# Autodesk Inventor assembly: WA673SA
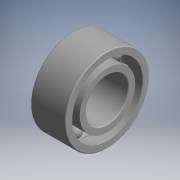
[picture p0: Inventor's stored thumbnail of the model, 180x180]
Saved by Autodesk Inventor 2017.3 (Build 213256000, 256)
## iProperties
Category: PARTsolutions
Company: NTN
Part Number: WA673SA
Catalog Web Link: www.cadenas.de
Description: With single shield Z-
Vendor: NTN
Document SubType Name: Assembly
Designer: partserver
Manufacturer: NTN
Mass: 0.0350333 g
Surface Area: 2.11591 cm^2
Volume: 0.0350333 cm^3
Density: 1 g/cm^3
Title: WA673SA
Author: Cadenas PARTsolutions
PSOL_IDENT_0: {$CADENAS_DATA\23d-libs\ntn\ball_roller_bearings\miniature_extra_small_bb\metric_system_sizes\mss_z_
PSOL_IDENT_1: asmtab.prj},185 {VTYP=3D},{STYP=ASSTAB},{NB=WA673SA},{LINA=WA673SA},{NN=With single shield Z},{DATE=
PSOL_IDENT_2: 21.12.2021 04:23:05},{GEOMDATE=10.03.2020 01:12:32},{VERSION=},{LINEID=11430},{WBVAR=},{WBNUMERIC=}
PSOL_IDENT_3: {NB=WA673SA},{LINA=WA673SA},{KT=DUMMY},{IDNR=},{SD=3.0},{D=6},{B=2.0},{B1=2.5},{D1=7.2},{D2=7.2},{C
PSOL_IDENT_4: 1=0.6},{C2=0.6},{R=0.08},{ORDER=WA673SA},{CR=268},{COR=94},{CU=2.47},{CRF=25},{CORF=9,5},{LSG=60 000
PSOL_IDENT_5: },{LSO=71 000},{MASS=0.20},{ORDER1=673},{WSS=WA673SA},{WDS=SSA},{UTWF=FL673},{FORSS=FLWA673SA},{FORD
PSOL_IDENT_6: S=SSA},{DA1=3,6},{DA2=4,1},{DA=5,4},{RAS=0,08},{MASS1=0.26},{VERS=2},{X=1.5},{N=9},{O=14.13},{RB=0.4
PSOL_IDENT_7: 44},{PPATH=mss_asmtpl.prj}
NB: WA673SA
NN: With single shield Z
NBSYN: $ORDER.
LINA: WA673SA
CATALOG: NTN Corporation
SD: 3
D: 6
B1: 2.5
R: 0.08
ORDER: WA673SA
CR: 268
COR: 94
CU: 2.47
LSG: 60 000
LSO: 71 000
MASS: 0.2
SUPPLIER: NTN
ARTICLENO: WA673SA
BOMINFO: WA673SA
CREATOR: CADENAS GmbH
## Documents named in this file (5)
- e:\temp\worker_43\temp\exporttempdir_1244_12_KYvLF\format_0\WA673SA.iam
- e:\temp\worker_43\temp\exporttempdir_1244_12_KYvLF\format_0\WA673SA Inner ring.ipt
- e:\temp\worker_43\temp\exporttempdir_1244_12_KYvLF\format_0\WA673SA Outer ring.ipt
- e:\temp\worker_43\temp\exporttempdir_1244_12_KYvLF\format_0\WA673SA Shield.ipt
- e:\temp\worker_43\temp\exporttempdir_1244_12_KYvLF\format_0\WA673SA Ball.ipt
## Components (12 placed, 4 different names)
1. WA673SA Inner ring:1 — mss_ir_Z@1 <-> mss_or_Z@2
2. WA673SA Outer ring:1 — mss_ir_Z@1 <-> mss_or_Z@2, mss_or11_XY@2 <-> mss_s_XY@3, mss_or11_Z@2 <-> mss_s_Z@3, mss_or11_YZ@2 <-> mss_s_YZ@3, mss_or21_1_XY@2 <-> mss_ball_XY@4, mss_or21_1_Z@2 <-> mss_ball_Z@4, mss_or21_1_YZ@2 <-> mss_ball_YZ@4, mss_or21_2_XY@2 <-> mss_ball_XY@5, mss_or21_2_Z@2 <-> mss_ball_Z@5, mss_or21_2_YZ@2 <-> mss_ball_YZ@5, mss_or21_3_XY@2 <-> mss_ball_XY@6, mss_or21_3_Z@2 <-> mss_ball_Z@6, mss_or21_3_YZ@2 <-> mss_ball_YZ@6, mss_or21_4_XY@2 <-> mss_ball_XY@7, mss_or21_4_Z@2 <-> mss_ball_Z@7, mss_or21_4_YZ@2 <-> mss_ball_YZ@7, mss_or21_5_XY@2 <-> mss_ball_XY@8, mss_or21_5_Z@2 <-> mss_ball_Z@8, mss_or21_5_YZ@2 <-> mss_ball_YZ@8, mss_or21_6_XY@2 <-> mss_ball_XY@9, mss_or21_6_Z@2 <-> mss_ball_Z@9, mss_or21_6_YZ@2 <-> mss_ball_YZ@9, mss_or21_7_XY@2 <-> mss_ball_XY@10, mss_or21_7_Z@2 <-> mss_ball_Z@10, mss_or21_7_YZ@2 <-> mss_ball_YZ@10, mss_or21_8_XY@2 <-> mss_ball_XY@11, mss_or21_8_Z@2 <-> mss_ball_Z@11, mss_or21_8_YZ@2 <-> mss_ball_YZ@11, mss_or21_9_XY@2 <-> mss_ball_XY@12, mss_or21_9_Z@2 <-> mss_ball_Z@12, mss_or21_9_YZ@2 <-> mss_ball_YZ@12
3. WA673SA Shield:1 — mss_or11_XY@2 <-> mss_s_XY@3, mss_or11_Z@2 <-> mss_s_Z@3, mss_or11_YZ@2 <-> mss_s_YZ@3
4. WA673SA Ball:1 — mss_or21_1_XY@2 <-> mss_ball_XY@4, mss_or21_1_Z@2 <-> mss_ball_Z@4, mss_or21_1_YZ@2 <-> mss_ball_YZ@4
5. WA673SA Ball:2 — mss_or21_2_XY@2 <-> mss_ball_XY@5, mss_or21_2_Z@2 <-> mss_ball_Z@5, mss_or21_2_YZ@2 <-> mss_ball_YZ@5
6. WA673SA Ball:3 — mss_or21_3_XY@2 <-> mss_ball_XY@6, mss_or21_3_Z@2 <-> mss_ball_Z@6, mss_or21_3_YZ@2 <-> mss_ball_YZ@6
7. WA673SA Ball:4 — mss_or21_4_XY@2 <-> mss_ball_XY@7, mss_or21_4_Z@2 <-> mss_ball_Z@7, mss_or21_4_YZ@2 <-> mss_ball_YZ@7
8. WA673SA Ball:5 — mss_or21_5_XY@2 <-> mss_ball_XY@8, mss_or21_5_Z@2 <-> mss_ball_Z@8, mss_or21_5_YZ@2 <-> mss_ball_YZ@8
9. WA673SA Ball:6 — mss_or21_6_XY@2 <-> mss_ball_XY@9, mss_or21_6_Z@2 <-> mss_ball_Z@9, mss_or21_6_YZ@2 <-> mss_ball_YZ@9
10. WA673SA Ball:7 — mss_or21_7_XY@2 <-> mss_ball_XY@10, mss_or21_7_Z@2 <-> mss_ball_Z@10, mss_or21_7_YZ@2 <-> mss_ball_YZ@10
11. WA673SA Ball:8 — mss_or21_8_XY@2 <-> mss_ball_XY@11, mss_or21_8_Z@2 <-> mss_ball_Z@11, mss_or21_8_YZ@2 <-> mss_ball_YZ@11
12. WA673SA Ball:9 — mss_or21_9_XY@2 <-> mss_ball_XY@12, mss_or21_9_Z@2 <-> mss_ball_Z@12, mss_or21_9_YZ@2 <-> mss_ball_YZ@12
## Relationships (31: Mate 20, Angle 10, Flush 1)
- mss_ir_Z@1 <-> mss_or_Z@2 [Mate]: WA673SA Inner ring:1 ↔ WA673SA Outer ring:1
- mss_or11_XY@2 <-> mss_s_XY@3 [Flush]: WA673SA Outer ring:1 ↔ WA673SA Shield:1
- mss_or11_Z@2 <-> mss_s_Z@3 [Mate]: WA673SA Outer ring:1 ↔ WA673SA Shield:1
- mss_or11_YZ@2 <-> mss_s_YZ@3 [Angle] (0 deg): WA673SA Outer ring:1 ↔ WA673SA Shield:1
- mss_or21_1_XY@2 <-> mss_ball_XY@4 [Mate]: WA673SA Outer ring:1 ↔ WA673SA Ball:1
- mss_or21_1_Z@2 <-> mss_ball_Z@4 [Mate]: WA673SA Outer ring:1 ↔ WA673SA Ball:1
- mss_or21_1_YZ@2 <-> mss_ball_YZ@4 [Angle] (0 deg): WA673SA Outer ring:1 ↔ WA673SA Ball:1
- mss_or21_2_XY@2 <-> mss_ball_XY@5 [Mate]: WA673SA Outer ring:1 ↔ WA673SA Ball:2
- mss_or21_2_Z@2 <-> mss_ball_Z@5 [Mate]: WA673SA Outer ring:1 ↔ WA673SA Ball:2
- mss_or21_2_YZ@2 <-> mss_ball_YZ@5 [Angle] (0 deg): WA673SA Outer ring:1 ↔ WA673SA Ball:2
- mss_or21_3_XY@2 <-> mss_ball_XY@6 [Mate]: WA673SA Outer ring:1 ↔ WA673SA Ball:3
- mss_or21_3_Z@2 <-> mss_ball_Z@6 [Mate]: WA673SA Outer ring:1 ↔ WA673SA Ball:3
- mss_or21_3_YZ@2 <-> mss_ball_YZ@6 [Angle] (0 deg): WA673SA Outer ring:1 ↔ WA673SA Ball:3
- mss_or21_4_XY@2 <-> mss_ball_XY@7 [Mate]: WA673SA Outer ring:1 ↔ WA673SA Ball:4
- mss_or21_4_Z@2 <-> mss_ball_Z@7 [Mate]: WA673SA Outer ring:1 ↔ WA673SA Ball:4
- mss_or21_4_YZ@2 <-> mss_ball_YZ@7 [Angle] (0 deg): WA673SA Outer ring:1 ↔ WA673SA Ball:4
- mss_or21_5_XY@2 <-> mss_ball_XY@8 [Mate]: WA673SA Outer ring:1 ↔ WA673SA Ball:5
- mss_or21_5_Z@2 <-> mss_ball_Z@8 [Mate]: WA673SA Outer ring:1 ↔ WA673SA Ball:5
- mss_or21_5_YZ@2 <-> mss_ball_YZ@8 [Angle] (0 deg): WA673SA Outer ring:1 ↔ WA673SA Ball:5
- mss_or21_6_XY@2 <-> mss_ball_XY@9 [Mate]: WA673SA Outer ring:1 ↔ WA673SA Ball:6
- mss_or21_6_Z@2 <-> mss_ball_Z@9 [Mate]: WA673SA Outer ring:1 ↔ WA673SA Ball:6
- mss_or21_6_YZ@2 <-> mss_ball_YZ@9 [Angle] (0 deg): WA673SA Outer ring:1 ↔ WA673SA Ball:6
- mss_or21_7_XY@2 <-> mss_ball_XY@10 [Mate]: WA673SA Outer ring:1 ↔ WA673SA Ball:7
- mss_or21_7_Z@2 <-> mss_ball_Z@10 [Mate]: WA673SA Outer ring:1 ↔ WA673SA Ball:7
- mss_or21_7_YZ@2 <-> mss_ball_YZ@10 [Angle] (0 deg): WA673SA Outer ring:1 ↔ WA673SA Ball:7
- mss_or21_8_XY@2 <-> mss_ball_XY@11 [Mate]: WA673SA Outer ring:1 ↔ WA673SA Ball:8
- mss_or21_8_Z@2 <-> mss_ball_Z@11 [Mate]: WA673SA Outer ring:1 ↔ WA673SA Ball:8
- mss_or21_8_YZ@2 <-> mss_ball_YZ@11 [Angle] (0 deg): WA673SA Outer ring:1 ↔ WA673SA Ball:8
- mss_or21_9_XY@2 <-> mss_ball_XY@12 [Mate]: WA673SA Outer ring:1 ↔ WA673SA Ball:9
- mss_or21_9_Z@2 <-> mss_ball_Z@12 [Mate]: WA673SA Outer ring:1 ↔ WA673SA Ball:9
- mss_or21_9_YZ@2 <-> mss_ball_YZ@12 [Angle] (0 deg): WA673SA Outer ring:1 ↔ WA673SA Ball:9
